# Autodesk Inventor assembly: ball_caster_full
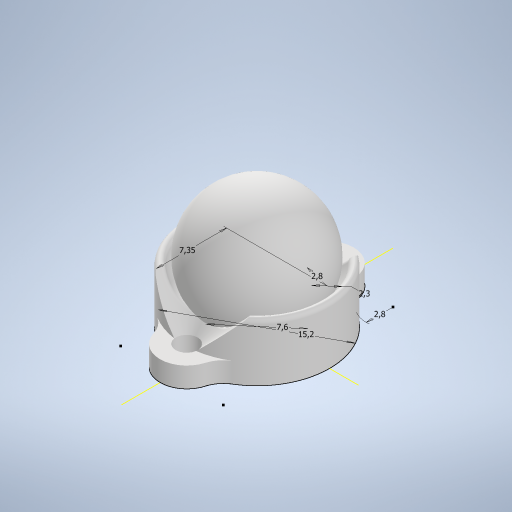
[picture p0: Inventor's stored thumbnail of the model, 512x512]
Saved by Autodesk Inventor 2024.3 (Build 283343000, 343)
## iProperties
Created: 2026-05-23
Part Number: ball_caster_full
Document SubType Name: Assembly
Designer: owozn
Author: owozn
## Documents named in this file (3)
- C:\Users\owozn\Documents\Nauka\Studia\mgr\Semestr_3\Magisterka\uMule\mechanics\subsets\ball_caster_full.iam
- C:\Users\owozn\Documents\Nauka\Studia\mgr\Semestr_3\Magisterka\uMule\mechanics\subsets\ball_caster.ipt
- C:\Users\owozn\Documents\Nauka\Studia\mgr\Semestr_3\Magisterka\uMule\mechanics\subsets\ball_for_caster.ipt
## Components (2 placed, 2 different names)
1. ball_caster:1 — Mate:1, Mate:2
2. ball_for_caster:1 — Mate:1, Mate:2
## Relationships (2: Mate 2)
- Mate:1: ball_caster:1 ↔ ball_for_caster:1
- Mate:2 (-6.35 mm): ball_caster:1 ↔ ball_for_caster:1
